# Autodesk Inventor assembly: bellows_kihon
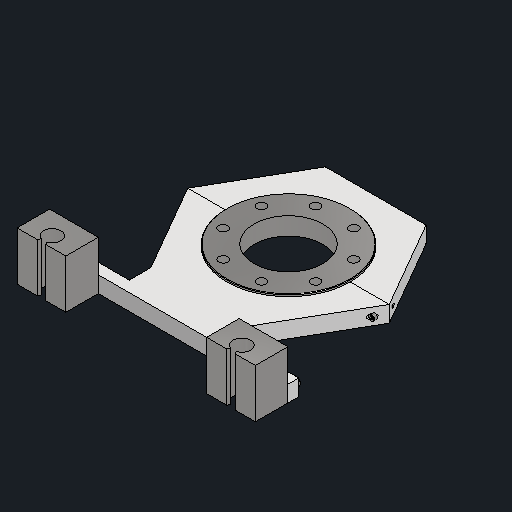
[picture p0: Inventor's stored thumbnail of the model, 512x512]
Saved by Autodesk Inventor 2027.1 (Build 311270010, 270A)
## iProperties
Created: 2026-06-03
Part Number: bellows_kihon
Document SubType Name: Assembly
Designer: shusu
Author: shusu
## Documents named in this file (7)
- C:\Users\queez\Dropbox\Drawings\PIHTI\bellows\bellows_1.iam
- C:\Users\queez\Dropbox\Drawings\PIHTI\bellows\bellows_flange.ipt
- C:\Users\queez\Dropbox\Drawings\PIHTI\bellows\flangeclamp_down.ipt
- C:\Users\queez\Dropbox\Drawings\PIHTI\bellows\flangeclamp_up.ipt
- C:\Users\queez\Dropbox\Drawings\PIHTI\ContentCenter\Fastners\JIS B 1176 - M3 x 16 - 0.5.ipt
- C:\Users\queez\Dropbox\Drawings\PIHTI\bellows\linearbearing.ipt
- C:\Users\queez\Dropbox\Drawings\PIHTI\ContentCenter\Fastners\JIS B 1176 - M5 x 16 - 0.8.ipt
## Components (11 placed, 6 different names)
1. bellows_flange:2 — Insert:4
2. flangeclamp_down:3 — Insert:4, Insert:10, Mate:6, Mate:8, Insert:13, Insert:14, Insert:17, Insert:18
3. flangeclamp_up:3 — Insert:8
4. JIS B 1176 - メートル M3 x 16:4 — Insert:8
5. JIS B 1176 - メートル M3 x 16:6 — Insert:10
6. linearbearing:2 — Mate:8
7. linearbearing:3 — Mate:6
8. JIS B 1176 - メートル M5 x 16:3 — Insert:13
9. JIS B 1176 - メートル M5 x 16:4 — Insert:14
10. JIS B 1176 - メートル M5 x 16:7 — Insert:18
11. JIS B 1176 - メートル M5 x 16:8 — Insert:17
## Relationships (11: Insert 7, Mate 4)
- [Mate]: flangeclamp_down:3 ↔ flangeclamp_up:3
- [Mate]: flangeclamp_down:3 ↔ flangeclamp_up:3
- Insert:4 (-15 mm): bellows_flange:2 ↔ flangeclamp_down:3
- Insert:8: flangeclamp_up:3 ↔ JIS B 1176 - メートル M3 x 16:4
- Insert:10: flangeclamp_down:3 ↔ JIS B 1176 - メートル M3 x 16:6
- Mate:6: flangeclamp_down:3 ↔ linearbearing:3
- Mate:8: flangeclamp_down:3 ↔ linearbearing:2
- Insert:13: flangeclamp_down:3 ↔ JIS B 1176 - メートル M5 x 16:3
- Insert:14: flangeclamp_down:3 ↔ JIS B 1176 - メートル M5 x 16:4
- Insert:17: flangeclamp_down:3 ↔ JIS B 1176 - メートル M5 x 16:8
- Insert:18: flangeclamp_down:3 ↔ JIS B 1176 - メートル M5 x 16:7
## Named parameters: d13_d11 = 0 mm, d14_d12 = 0 mm
